# Autodesk Inventor assembly: Linear Actuator_CPY
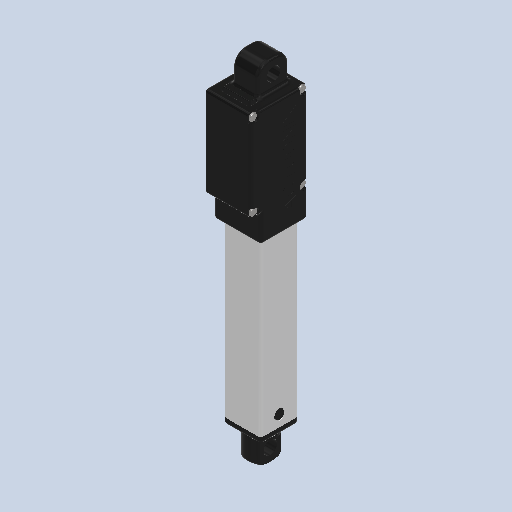
[picture p0: Inventor's stored thumbnail of the model, 512x512]
Saved by Autodesk Inventor 2024.1 (Build 281209000, 209)
## iProperties
Created: 2016-10-05
Part Number: Linear Actuator_CPY
Document SubType Name: Assembly
Designer: udayk
Title: L12_50MM_ASM
Author: Mike
Revision Number: 1LAST_VERSION
## Documents named in this file (10)
- C:\Users\udayk\OneDrive\Desktop\Year 1\Engineer IP13\Project 3\Thurs-08 Modelling\2. Hopper Assembly\2. Hopper Assembly\Linear Actuator_CPY.iam
- C:\Users\udayk\OneDrive\Desktop\Year 1\Engineer IP13\Project 3\Thurs-08 Modelling\2. Hopper Assembly\2. Hopper Assembly\EXTENSION_10404_50MM_CPY.ipt
- C:\Users\udayk\OneDrive\Desktop\Year 1\Engineer IP13\Project 3\Thurs-08 Modelling\2. Hopper Assembly\2. Hopper Assembly\CLAMSHELL_BOT_10417_CPY.ipt
- C:\Users\udayk\OneDrive\Desktop\Year 1\Engineer IP13\Project 3\Thurs-08 Modelling\2. Hopper Assembly\2. Hopper Assembly\CLAMSHELL_TOP_10416_CPY.ipt
- C:\Users\udayk\OneDrive\Desktop\Year 1\Engineer IP13\Project 3\Thurs-08 Modelling\2. Hopper Assembly\2. Hopper Assembly\FASTENER_10427_CPY.ipt
- C:\Users\udayk\OneDrive\Desktop\Year 1\Engineer IP13\Project 3\Thurs-08 Modelling\2. Hopper Assembly\2. Hopper Assembly\GUIDE_10429_CPY.ipt
- C:\Users\udayk\OneDrive\Desktop\Year 1\Engineer IP13\Project 3\Thurs-08 Modelling\2. Hopper Assembly\2. Hopper Assembly\NUT_10419_CPY.ipt
- C:\Users\udayk\OneDrive\Desktop\Year 1\Engineer IP13\Project 3\Thurs-08 Modelling\2. Hopper Assembly\2. Hopper Assembly\SHAFT_10409_50MM_CPY.ipt
- C:\Users\udayk\OneDrive\Desktop\Year 1\Engineer IP13\Project 3\Thurs-08 Modelling\2. Hopper Assembly\2. Hopper Assembly\PLUG_10428_CPY.ipt
- C:\Users\udayk\OneDrive\Desktop\Year 1\Engineer IP13\Project 3\Thurs-08 Modelling\2. Hopper Assembly\2. Hopper Assembly\GROMMET_3_HOLE_CPY.ipt
## Components (12 placed, 9 different names)
1. EXTENSION_10404_50MM_CPYmover:1 — Mate:20, Mate:19, Mate:18, Flush:2, Angle:7, Mate:23, Angle:8
2. CLAMSHELL_BOT_10417_CPYmover:1 — Mate:20, Mate:19, Mate:18, Mate:9, Mate:8, Mate:7, Angle:4, Mate:1, Angle:1, Mate:4, Angle:2, Mate:3, Angle:3, Mate:2, Mate:26, Angle:5, Mate:15, Angle:6, Flush:1, Mate:6, Mate:5
3. CLAMSHELL_TOP_10416_CPYmover:1 — Mate:9, Mate:8, Mate:7, Mate:13, Mate:12, Mate:11, Mate:10
4. FASTENER_10427_CPYmover:1 — Mate:13, Angle:4, Mate:1
5. FASTENER_10427_CPYmover:2 — Mate:12, Angle:1, Mate:4
6. FASTENER_10427_CPYmover:3 — Mate:11, Angle:2, Mate:3
7. FASTENER_10427_CPYmover:4 — Mate:10, Angle:3, Mate:2
8. GUIDE_10429_CPYmover:1 — Flush:2, Angle:7, Mate:23
9. NUT_10419_CPYmover:1 — Mate:26, Angle:5, Mate:15, Mate:22, Mate:21
10. SHAFT_10409_50MM_CPYmover:1 — Mate:22, Angle:6, Mate:21, Mate:25, Mate:24
11. PLUG_10428_CPYmover:1 — Angle:8, Mate:25, Mate:24
12. GROMMET_3_HOLE_CPYmover:1 — Flush:1, Mate:6, Mate:5
## Relationships (33: Mate 23, Angle 8, Flush 2)
- Mate:20: EXTENSION_10404_50MM_CPYmover:1 ↔ CLAMSHELL_BOT_10417_CPYmover:1
- Mate:19: EXTENSION_10404_50MM_CPYmover:1 ↔ CLAMSHELL_BOT_10417_CPYmover:1
- Mate:18: EXTENSION_10404_50MM_CPYmover:1 ↔ CLAMSHELL_BOT_10417_CPYmover:1
- Mate:9: CLAMSHELL_BOT_10417_CPYmover:1 ↔ CLAMSHELL_TOP_10416_CPYmover:1
- Mate:8: CLAMSHELL_BOT_10417_CPYmover:1 ↔ CLAMSHELL_TOP_10416_CPYmover:1
- Mate:7: CLAMSHELL_BOT_10417_CPYmover:1 ↔ CLAMSHELL_TOP_10416_CPYmover:1
- Mate:13: CLAMSHELL_TOP_10416_CPYmover:1 ↔ FASTENER_10427_CPYmover:1
- Angle:4 (0 deg): CLAMSHELL_BOT_10417_CPYmover:1 ↔ FASTENER_10427_CPYmover:1
- Mate:1: CLAMSHELL_BOT_10417_CPYmover:1 ↔ FASTENER_10427_CPYmover:1
- Mate:12: CLAMSHELL_TOP_10416_CPYmover:1 ↔ FASTENER_10427_CPYmover:2
- Angle:1 (0 deg): CLAMSHELL_BOT_10417_CPYmover:1 ↔ FASTENER_10427_CPYmover:2
- Mate:4: CLAMSHELL_BOT_10417_CPYmover:1 ↔ FASTENER_10427_CPYmover:2
- Mate:11: CLAMSHELL_TOP_10416_CPYmover:1 ↔ FASTENER_10427_CPYmover:3
- Angle:2 (0 deg): CLAMSHELL_BOT_10417_CPYmover:1 ↔ FASTENER_10427_CPYmover:3
- Mate:3: CLAMSHELL_BOT_10417_CPYmover:1 ↔ FASTENER_10427_CPYmover:3
- Mate:10: CLAMSHELL_TOP_10416_CPYmover:1 ↔ FASTENER_10427_CPYmover:4
- Angle:3 (0 deg): CLAMSHELL_BOT_10417_CPYmover:1 ↔ FASTENER_10427_CPYmover:4
- Mate:2: CLAMSHELL_BOT_10417_CPYmover:1 ↔ FASTENER_10427_CPYmover:4
- Flush:2: EXTENSION_10404_50MM_CPYmover:1 ↔ GUIDE_10429_CPYmover:1
- Angle:7 (0 deg): EXTENSION_10404_50MM_CPYmover:1 ↔ GUIDE_10429_CPYmover:1
- Mate:23: EXTENSION_10404_50MM_CPYmover:1 ↔ GUIDE_10429_CPYmover:1
- Mate:26: CLAMSHELL_BOT_10417_CPYmover:1 ↔ NUT_10419_CPYmover:1
- Angle:5 (270 deg): CLAMSHELL_BOT_10417_CPYmover:1 ↔ NUT_10419_CPYmover:1
- Mate:15: CLAMSHELL_BOT_10417_CPYmover:1 ↔ NUT_10419_CPYmover:1
- Mate:22: NUT_10419_CPYmover:1 ↔ SHAFT_10409_50MM_CPYmover:1
- Angle:6 (0 deg): CLAMSHELL_BOT_10417_CPYmover:1 ↔ SHAFT_10409_50MM_CPYmover:1
- Mate:21: NUT_10419_CPYmover:1 ↔ SHAFT_10409_50MM_CPYmover:1
- Angle:8 (0 deg): EXTENSION_10404_50MM_CPYmover:1 ↔ PLUG_10428_CPYmover:1
- Mate:25: SHAFT_10409_50MM_CPYmover:1 ↔ PLUG_10428_CPYmover:1
- Mate:24: SHAFT_10409_50MM_CPYmover:1 ↔ PLUG_10428_CPYmover:1
- Flush:1 (0.936 mm): CLAMSHELL_BOT_10417_CPYmover:1 ↔ GROMMET_3_HOLE_CPYmover:1
- Mate:6: CLAMSHELL_BOT_10417_CPYmover:1 ↔ GROMMET_3_HOLE_CPYmover:1
- Mate:5 (0.25 mm): CLAMSHELL_BOT_10417_CPYmover:1 ↔ GROMMET_3_HOLE_CPYmover:1
